# Autodesk Inventor assembly: BG103_trajan20_22
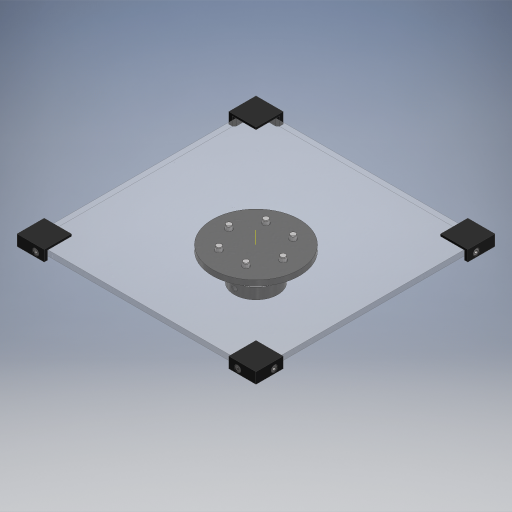
[picture p0: Inventor's stored thumbnail of the model, 512x512]
Saved by Autodesk Inventor 2023 (Build 270158000, 158)
## iProperties
Company: HTBLA Kaindorf
RuleStatus: InUse
Created: 2022-11-06
Part Number: BG103_trajan20_22
Project: Zeichenmaschine_neu
Material: Generisch
Description: Papierplatte
Document SubType Name: Assembly
Designer: trajan20
AfterDocNew0: iProperties-Editor_aufrufen
Author: jan
Keywords: 2022
## Documents named in this file (6)
- C:\Users\jan\Documents\Zeichenmaschine_neu\BG103_trajan20_22_Zeichenmaschine_neu_Papierplatte.iam
- C:\Users\jan\Documents\Zeichenmaschine_neu\BT403_trajan20_21_Zeichenmaschine_v2_papierplatte_plexi.ipt
- C:\Users\jan\Documents\Zeichenmaschine_neu\BT405_trajan20_21_Zeichenmaschine_v2_zwischenteil_stifte.ipt
- C:\Users\jan\Documents\Zeichenmaschine_neu\BT406_trajan20_21_Zeichenmaschine_v2_Ecken.ipt
- C:\Users\jan\Documents\Zeichenmaschine_neu\Normteile\de-DE\ISO 2338(1)\DIN EN ISO 2338 - 5 h8 x 16.ipt
- C:\Users\jan\Documents\Zeichenmaschine_neu\Normteile\de-DE\ISO 4762(2)\ISO 4762 - M3 x 8ISO.ipt
## Components (20 placed, 5 different names)
1. BT403_trajan20_21_Zeichenmaschine_v2_papierplatte_plexi:1 — Passend:1, Passend:2, Passend:3, Passend:16, Passend:17, Passend:18, Passend:19, Passend:20, Passend:21, Passend:22, Passend:23, Passend:24, Passend:25, Passend:26, Passend:27
2. DIN EN ISO 2338 5 h8 x 16:1 — Passend:4, Passend:11
3. DIN EN ISO 2338 5 h8 x 16:2 — Passend:5, Passend:10
4. DIN EN ISO 2338 5 h8 x 16:3 — Passend:6, Passend:15
5. DIN EN ISO 2338 5 h8 x 16:4 — Passend:7, Passend:14
6. DIN EN ISO 2338 5 h8 x 16:5 — Passend:8, Passend:13
7. DIN EN ISO 2338 5 h8 x 16:6 — Passend:9, Passend:12
8. BT405_trajan20_21_Zeichenmaschine_v2_zwischenteil_stifte:1 — Passend:1, Passend:2, Passend:3, Passend:4, Passend:5, Passend:6, Passend:7, Passend:8, Passend:9, Passend:10, Passend:11, Passend:12, Passend:13, Passend:14, Passend:15
9. BT406_trajan20_21_Zeichenmaschine_v2_Ecken:1 — Passend:16, Passend:17, Passend:18, Einfügen:6, Einfügen:8
10. BT406_trajan20_21_Zeichenmaschine_v2_Ecken:2 — Passend:19, Passend:20, Passend:21, Einfügen:2, Einfügen:4
11. BT406_trajan20_21_Zeichenmaschine_v2_Ecken:3 — Passend:22, Passend:23, Passend:24, Einfügen:1, Einfügen:7
12. BT406_trajan20_21_Zeichenmaschine_v2_Ecken:4 — Passend:25, Passend:26, Passend:27, Einfügen:3, Einfügen:5
13. ISO 4762 M3 x 8:1 — Einfügen:1
14. ISO 4762 M3 x 8:2 — Einfügen:2
15. ISO 4762 M3 x 8:3 — Einfügen:3
16. ISO 4762 M3 x 8:4 — Einfügen:4
17. ISO 4762 M3 x 8:5 — Einfügen:5
18. ISO 4762 M3 x 8:6 — Einfügen:6
19. ISO 4762 M3 x 8:7 — Einfügen:7
20. ISO 4762 M3 x 8:8 — Einfügen:8
## Relationships (35: Mate 27, Insert 8)
- Passend:1 [Mate]: BT403_trajan20_21_Zeichenmaschine_v2_papierplatte_plexi:1 ↔ BT405_trajan20_21_Zeichenmaschine_v2_zwischenteil_stifte:1
- Passend:2 [Mate]: BT403_trajan20_21_Zeichenmaschine_v2_papierplatte_plexi:1 ↔ BT405_trajan20_21_Zeichenmaschine_v2_zwischenteil_stifte:1
- Passend:3 [Mate]: BT403_trajan20_21_Zeichenmaschine_v2_papierplatte_plexi:1 ↔ BT405_trajan20_21_Zeichenmaschine_v2_zwischenteil_stifte:1
- Passend:4 [Mate]: DIN EN ISO 2338 5 h8 x 16:1 ↔ BT405_trajan20_21_Zeichenmaschine_v2_zwischenteil_stifte:1
- Passend:5 [Mate]: DIN EN ISO 2338 5 h8 x 16:2 ↔ BT405_trajan20_21_Zeichenmaschine_v2_zwischenteil_stifte:1
- Passend:6 [Mate]: DIN EN ISO 2338 5 h8 x 16:3 ↔ BT405_trajan20_21_Zeichenmaschine_v2_zwischenteil_stifte:1
- Passend:7 [Mate]: DIN EN ISO 2338 5 h8 x 16:4 ↔ BT405_trajan20_21_Zeichenmaschine_v2_zwischenteil_stifte:1
- Passend:8 [Mate]: DIN EN ISO 2338 5 h8 x 16:5 ↔ BT405_trajan20_21_Zeichenmaschine_v2_zwischenteil_stifte:1
- Passend:9 [Mate]: DIN EN ISO 2338 5 h8 x 16:6 ↔ BT405_trajan20_21_Zeichenmaschine_v2_zwischenteil_stifte:1
- Passend:10 [Mate]: DIN EN ISO 2338 5 h8 x 16:2 ↔ BT405_trajan20_21_Zeichenmaschine_v2_zwischenteil_stifte:1
- Passend:11 [Mate]: DIN EN ISO 2338 5 h8 x 16:1 ↔ BT405_trajan20_21_Zeichenmaschine_v2_zwischenteil_stifte:1
- Passend:12 [Mate]: DIN EN ISO 2338 5 h8 x 16:6 ↔ BT405_trajan20_21_Zeichenmaschine_v2_zwischenteil_stifte:1
- Passend:13 [Mate]: DIN EN ISO 2338 5 h8 x 16:5 ↔ BT405_trajan20_21_Zeichenmaschine_v2_zwischenteil_stifte:1
- Passend:14 [Mate]: DIN EN ISO 2338 5 h8 x 16:4 ↔ BT405_trajan20_21_Zeichenmaschine_v2_zwischenteil_stifte:1
- Passend:15 [Mate]: DIN EN ISO 2338 5 h8 x 16:3 ↔ BT405_trajan20_21_Zeichenmaschine_v2_zwischenteil_stifte:1
- Passend:16 [Mate]: BT403_trajan20_21_Zeichenmaschine_v2_papierplatte_plexi:1 ↔ BT406_trajan20_21_Zeichenmaschine_v2_Ecken:1
- Passend:17 [Mate]: BT403_trajan20_21_Zeichenmaschine_v2_papierplatte_plexi:1 ↔ BT406_trajan20_21_Zeichenmaschine_v2_Ecken:1
- Passend:18 [Mate] (1.5 mm): BT403_trajan20_21_Zeichenmaschine_v2_papierplatte_plexi:1 ↔ BT406_trajan20_21_Zeichenmaschine_v2_Ecken:1
- Passend:19 [Mate]: BT403_trajan20_21_Zeichenmaschine_v2_papierplatte_plexi:1 ↔ BT406_trajan20_21_Zeichenmaschine_v2_Ecken:2
- Passend:20 [Mate]: BT403_trajan20_21_Zeichenmaschine_v2_papierplatte_plexi:1 ↔ BT406_trajan20_21_Zeichenmaschine_v2_Ecken:2
- Passend:21 [Mate] (1.5 mm): BT403_trajan20_21_Zeichenmaschine_v2_papierplatte_plexi:1 ↔ BT406_trajan20_21_Zeichenmaschine_v2_Ecken:2
- Passend:22 [Mate]: BT403_trajan20_21_Zeichenmaschine_v2_papierplatte_plexi:1 ↔ BT406_trajan20_21_Zeichenmaschine_v2_Ecken:3
- Passend:23 [Mate]: BT403_trajan20_21_Zeichenmaschine_v2_papierplatte_plexi:1 ↔ BT406_trajan20_21_Zeichenmaschine_v2_Ecken:3
- Passend:24 [Mate] (1.5 mm): BT403_trajan20_21_Zeichenmaschine_v2_papierplatte_plexi:1 ↔ BT406_trajan20_21_Zeichenmaschine_v2_Ecken:3
- Passend:25 [Mate]: BT403_trajan20_21_Zeichenmaschine_v2_papierplatte_plexi:1 ↔ BT406_trajan20_21_Zeichenmaschine_v2_Ecken:4
- Passend:26 [Mate]: BT403_trajan20_21_Zeichenmaschine_v2_papierplatte_plexi:1 ↔ BT406_trajan20_21_Zeichenmaschine_v2_Ecken:4
- Passend:27 [Mate] (1.5 mm): BT403_trajan20_21_Zeichenmaschine_v2_papierplatte_plexi:1 ↔ BT406_trajan20_21_Zeichenmaschine_v2_Ecken:4
- Einfügen:1 [Insert]: BT406_trajan20_21_Zeichenmaschine_v2_Ecken:3 ↔ ISO 4762 M3 x 8:1
- Einfügen:2 [Insert]: BT406_trajan20_21_Zeichenmaschine_v2_Ecken:2 ↔ ISO 4762 M3 x 8:2
- Einfügen:3 [Insert]: BT406_trajan20_21_Zeichenmaschine_v2_Ecken:4 ↔ ISO 4762 M3 x 8:3
- Einfügen:4 [Insert]: BT406_trajan20_21_Zeichenmaschine_v2_Ecken:2 ↔ ISO 4762 M3 x 8:4
- Einfügen:5 [Insert]: BT406_trajan20_21_Zeichenmaschine_v2_Ecken:4 ↔ ISO 4762 M3 x 8:5
- Einfügen:6 [Insert]: BT406_trajan20_21_Zeichenmaschine_v2_Ecken:1 ↔ ISO 4762 M3 x 8:6
- Einfügen:7 [Insert]: BT406_trajan20_21_Zeichenmaschine_v2_Ecken:3 ↔ ISO 4762 M3 x 8:7
- Einfügen:8 [Insert]: BT406_trajan20_21_Zeichenmaschine_v2_Ecken:1 ↔ ISO 4762 M3 x 8:8
